# Autodesk Inventor assembly: S2x1
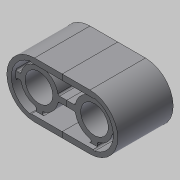
[picture p0: Inventor's stored thumbnail of the model, 180x180]
Saved by Autodesk Inventor 2020 (Build 240168000, 168)
## iProperties
Created: 2019-04-27
Part Number: S2x1
Document SubType Name: Assembly
Designer: Varga Daniel
Author: Varga Daniel
## Documents named in this file (3)
- C:\!_Dani\!_cloud\OneDrive\!_munka\Revolution\StructuralParts\Beams\Straight Beams\S1+x1\S2x1.iam
- C:\!_Dani\!_cloud\OneDrive\!_munka\Revolution\StructuralParts\Beams\beam_single_end_part.ipt
- C:\!_Dani\!_cloud\OneDrive\!_munka\Revolution\StructuralParts\Beams\Straight Beams\S1+x1.iam
## Components (2 placed, 1 different names)
1. beam_single_end_part:1 — Flush:1, Flush:2, Flush:3, Flush:4, End_part_mate, Flush:5
2. beam_single_end_part:2 — Flush:4, End_part_mate, Flush:5
## Relationships (6: Flush 5, Mate 1)
- Flush:1: beam_single_end_part:1
- Flush:2: beam_single_end_part:1
- Flush:3: beam_single_end_part:1
- Flush:4: beam_single_end_part:1 ↔ beam_single_end_part:2
- End_part_mate [Mate]: beam_single_end_part:1 ↔ beam_single_end_part:2
- Flush:5: beam_single_end_part:1 ↔ beam_single_end_part:2
